# Autodesk Inventor assembly: handle
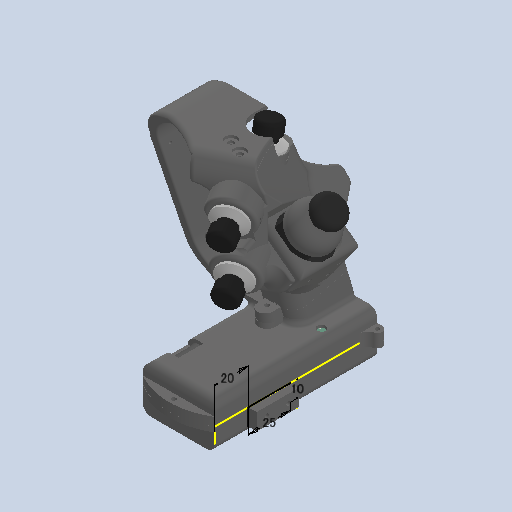
[picture p0: Inventor's stored thumbnail of the model, 512x512]
Saved by Autodesk Inventor 2026.1 (Build 301233020, 233B)
## iProperties
Created: 2026-01-22
Part Number: handle
Document SubType Name: Assembly
Designer: hibik
Author: hibik
## Documents named in this file (7)
- C:\Users\hibik\Documents\Robomech\HR\controller\hard\handle_right\handle.iam
- C:\Users\hibik\Documents\Robomech\HR\controller\hard\handle_right\handle_outside.ipt
- C:\Users\hibik\Documents\Robomech\HR\controller\hard\handle_right\pannel_push_sw.ipt
- C:\Users\hibik\Documents\Robomech\HR\controller\hard\handle_right\handle_inside.ipt
- C:\Users\hibik\Documents\Robomech\HR\controller\hard\handle_right\handle_monitor.iam
- C:\Users\hibik\Documents\Robomech\HR\controller\hard\handle_right\handle_inside_cover.ipt
- C:\Users\hibik\Documents\Robomech\HR\controller\hard\handle_right\stick.ipt
## Components (8 placed, 6 different names)
1. handle_outside:1 — フラッシュ:1, フラッシュ:2, フラッシュ:3, メイト:1, フラッシュ:4
2. pannel_push_sw:1
3. pannel_push_sw:2
4. pannel_push_sw:3
5. handle_inside:1 — フラッシュ:1, フラッシュ:2, フラッシュ:3, メイト:1, フラッシュ:4, メイト:2, メイト:3, メイト:4
6. handle_monitor:1 [sub-assembly]
7. handle_inside_cover:1
8. stick:1 — メイト:2, メイト:3, メイト:4
## Relationships (8: Flush 4, Mate 4)
- フラッシュ:1 [Flush]: handle_outside:1 ↔ handle_inside:1
- フラッシュ:2 [Flush]: handle_outside:1 ↔ handle_inside:1
- フラッシュ:3 [Flush]: handle_outside:1 ↔ handle_inside:1
- メイト:1 [Mate]: handle_outside:1 ↔ handle_inside:1
- フラッシュ:4 [Flush]: handle_outside:1 ↔ handle_inside:1
- メイト:2 [Mate]: handle_inside:1 ↔ stick:1
- メイト:3 [Mate]: handle_inside:1 ↔ stick:1
- メイト:4 [Mate]: handle_inside:1 ↔ stick:1
